# Autodesk Inventor assembly: z_assembly
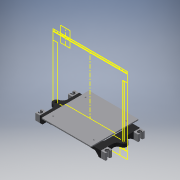
[picture p0: Inventor's stored thumbnail of the model, 180x180]
Saved by Autodesk Inventor 2016 (Build 200138000, 138)
## iProperties
Created: 2016-06-30
Part Number: z_assembly
Document SubType Name: Assembly
Designer: brent
Author: brent
## Documents named in this file (3)
- C:\Users\brent\OneDrive\personal\printer_cad\z_assembly.iam
- C:\Users\brent\OneDrive\personal\printer_cad\zaxis.ipt
- C:\Users\brent\OneDrive\personal\printer_cad\offtheshelf\sbr12uu.ipt
## Components (5 placed, 2 different names)
1. zaxis:1 — Mate:1, Mate:2, Mate:3, Mate:4, Mate:5, Mate:6, Mate:7, Mate:8
2. sbr12uu:1 — Mate:1, Mate:2
3. sbr12uu:2 — Mate:3, Mate:4
4. sbr12uu:3 — Mate:5, Mate:6
5. sbr12uu:4 — Mate:7, Mate:8
## Relationships (8: Mate 8)
- Mate:1: zaxis:1 ↔ sbr12uu:1
- Mate:2: zaxis:1 ↔ sbr12uu:1
- Mate:3: zaxis:1 ↔ sbr12uu:2
- Mate:4: zaxis:1 ↔ sbr12uu:2
- Mate:5: zaxis:1 ↔ sbr12uu:3
- Mate:6: zaxis:1 ↔ sbr12uu:3
- Mate:7: zaxis:1 ↔ sbr12uu:4
- Mate:8: zaxis:1 ↔ sbr12uu:4
